# Autodesk Inventor assembly: DribblerUnit
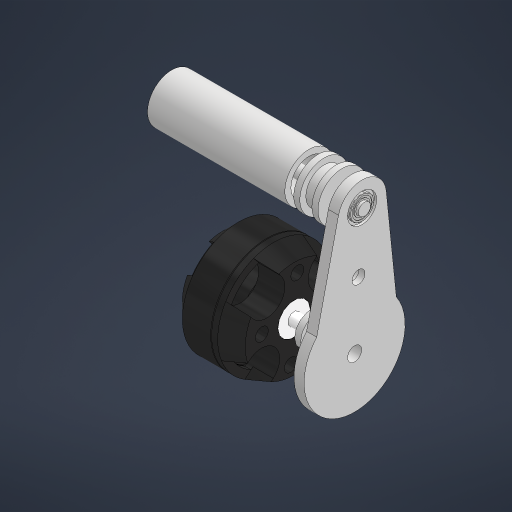
[picture p0: Inventor's stored thumbnail of the model, 512x512]
Saved by Autodesk Inventor 2024.2 (Build 282272000, 272)
## iProperties
Created: 2023-12-27
Part Number: DribblerUnit
Document SubType Name: Assembly
Designer: Hanaoka
Author: Hanaoka
## Documents named in this file (8)
- G:\共有ドライブ\reRo\05_個人\hanaoka\inventor\DribblerUnit\DribblerUnit.iam
- G:\共有ドライブ\reRo\05_個人\hanaoka\inventor\DribblerUnit\C2822_BLDC.ipt
- G:\共有ドライブ\reRo\05_個人\hanaoka\inventor\DribblerUnit\Shaft_D3.ipt
- G:\共有ドライブ\reRo\05_個人\hanaoka\inventor\DribblerUnit\tube.ipt
- G:\共有ドライブ\reRo\05_個人\hanaoka\inventor\DribblerUnit\Bearing_C-FL673ZZ.ipt
- G:\共有ドライブ\reRo\05_個人\hanaoka\inventor\DribblerUnit\Main_Frame.ipt
- G:\共有ドライブ\reRo\05_個人\hanaoka\inventor\DribblerUnit\Pulley_D3_P6.ipt
- G:\共有ドライブ\reRo\05_個人\hanaoka\inventor\DribblerUnit\Pulley_D3_P10.ipt
## Components (7 placed, 7 different names)
1. C2822_BLDC:1 — 挿入:4, メイト:10
2. Main_Frame:1 — メイト:2, 正接:1, 挿入:4, メイト:5, メイト:6
3. Pulley_D3_P10:1 — メイト:8
4. tube:1 — メイト:9
5. Shaft_D3:1 — メイト:7, メイト:8, メイト:9
6. Bearing_C-FL673ZZ:1 — メイト:5, メイト:6, メイト:7
7. Pulley_D3_P6:1 — メイト:10
## Relationships (9: Mate 7, Tangent 1, Insert 1)
- メイト:2 [Mate]: Main_Frame:1
- 正接:1 [Tangent]: Main_Frame:1
- 挿入:4 [Insert]: C2822_BLDC:1 ↔ Main_Frame:1
- メイト:5 [Mate]: Main_Frame:1 ↔ Bearing_C-FL673ZZ:1
- メイト:6 [Mate]: Main_Frame:1 ↔ Bearing_C-FL673ZZ:1
- メイト:7 [Mate]: Shaft_D3:1 ↔ Bearing_C-FL673ZZ:1
- メイト:8 [Mate]: Pulley_D3_P10:1 ↔ Shaft_D3:1
- メイト:9 [Mate]: tube:1 ↔ Shaft_D3:1
- メイト:10 [Mate]: C2822_BLDC:1 ↔ Pulley_D3_P6:1
